# Autodesk Inventor assembly: linear_actuator_as
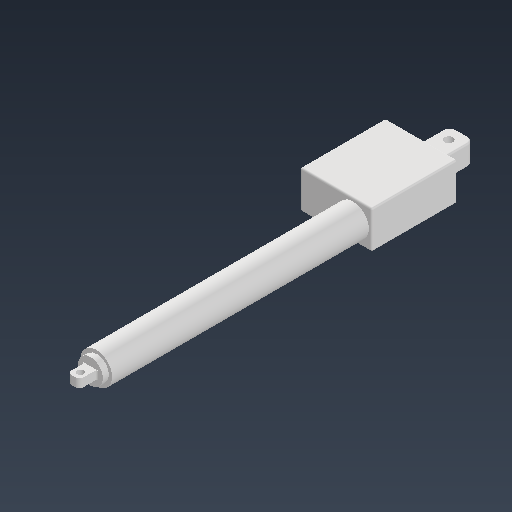
[picture p0: Inventor's stored thumbnail of the model, 512x512]
Saved by Autodesk Inventor 2021 (Build 250183000, 183)
## iProperties
Created: 2021-06-25
Part Number: linear_actuator_as
Document SubType Name: Assembly
## Documents named in this file (3)
- C:\Users\Watchdog\OneDrive - Flinders\Advn Mech Design Shared\6_Development\2_Design\inventor\cover\linear_actuator_as.iam
- C:\Users\Watchdog\OneDrive - Flinders\Advn Mech Design Shared\6_Development\2_Design\inventor\cover\linear_actuator_LH.ipt
- C:\Users\Watchdog\OneDrive - Flinders\Advn Mech Design Shared\6_Development\2_Design\inventor\cover\linear_actuator_SH.ipt
## Components (2 placed, 2 different names)
1. linear_actuator_LH:1 — Mate:1, Mate:2, Flush:1, Mate:3, Mate:4
2. linear_actuator_SH:1 — Mate:3, Mate:4
## Relationships (5: Mate 4, Flush 1)
- Mate:1: linear_actuator_LH:1
- Mate:2: linear_actuator_LH:1
- Flush:1: linear_actuator_LH:1
- Mate:3: linear_actuator_LH:1 ↔ linear_actuator_SH:1
- Mate:4: linear_actuator_LH:1 ↔ linear_actuator_SH:1
